# Autodesk Inventor assembly: Bearing Block Assembly
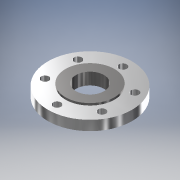
[picture p0: Inventor's stored thumbnail of the model, 180x180]
Saved by Autodesk Inventor 2019.4 (Build 234330000, 330)
## iProperties
Created: 2020-01-05
Part Number: Bearing Block Assembly
Document SubType Name: Assembly
Designer: Mark
Mass: 70.7644 g
Surface Area: 92.0879 cm^2
Volume: 17.567 cm^3
Density: 4.02826 g/cm^3
Author: Mark
## Documents named in this file (3)
- C:\Users\Mark\Desktop\7738 Helion Engineering\7738-2020\CAD\Bearing Block Assembly.iam
- C:\Users\Mark\Desktop\7738 Helion Engineering\7738-2020\CAD\Bearing Block.ipt
- C:\Users\Mark\Desktop\7738 Helion Engineering\7738-2020\CAD\F6804zz.ipt
## Components (2 placed, 2 different names)
1. Bearing Block:1 — Mate:1, Mate:2
2. F6804zz:1 — Mate:1, Mate:2
## Relationships (2: Mate 2)
- Mate:1: Bearing Block:1 ↔ F6804zz:1
- Mate:2: Bearing Block:1 ↔ F6804zz:1
